# Autodesk Inventor assembly: GIM8108-8
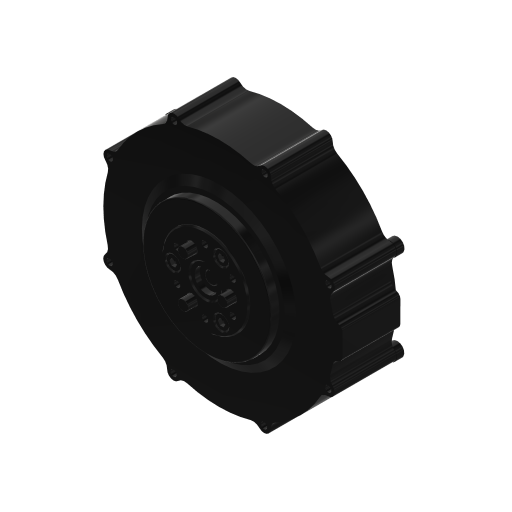
[picture p0: Inventor's stored thumbnail of the model, 512x512]
Saved by Autodesk Inventor 2023 (Build 270158000, 158)
## iProperties
Created: 2024-11-05
Part Number: GIM8108-8
Document SubType Name: Assembly
Designer: kiyo
Mass: 396 g
Surface Area: 491.411 cm^2
Volume: 132.201 cm^3
Author: kiyo
## Documents named in this file (3)
- D:\GitHub\inventor\syu-si\OfficeRobot\ReadyMade\Steadywin\GIM8108-8.iam
- D:\GitHub\inventor\syu-si\OfficeRobot\ReadyMade\Steadywin\GIM8108-8_1.ipt
- D:\GitHub\inventor\syu-si\OfficeRobot\ReadyMade\Steadywin\GIM8108-8_2.ipt
## Components (2 placed, 2 different names)
1. GIM8108-8_1:1 — 挿入:1
2. GIM8108-8_2:1 — 挿入:1, 角度:1
## Relationships (2: Insert 1, Angle 1)
- 挿入:1 [Insert]: GIM8108-8_1:1 ↔ GIM8108-8_2:1
- 角度:1 [Angle] (90 deg): GIM8108-8_2:1
